# Autodesk Inventor assembly: WheelFront
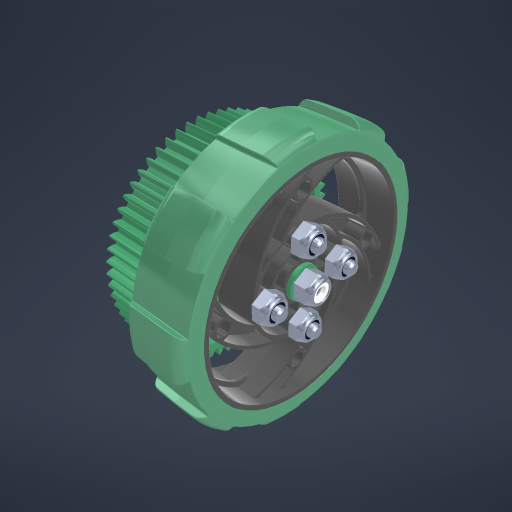
[picture p0: Inventor's stored thumbnail of the model, 512x512]
Saved by Autodesk Inventor 2023 (Build 270158000, 158)
## iProperties
Created: 2022-08-31
Part Number: WheelFront
Document SubType Name: Assembly
Designer: alex
Author: alex
## Documents named in this file (12)
- C:\Users\alex\Documents\GitHub\4067X_spin_up_cad\Chassis\TractionCentre.iam
- C:\Users\alex\Documents\GitHub\4067X_spin_up_cad\Library\Motion\Spacers\Spacer Nylon .375 OD.ipt
- C:\Users\alex\Documents\GitHub\4067X_spin_up_cad\Library\Structure\Hardware\Nut Keps.ipt
- C:\Users\alex\Documents\GitHub\4067X_spin_up_cad\Library\Structure\Hardware\Nut Nylock.ipt
- C:\Users\alex\Documents\GitHub\4067X_spin_up_cad\Library\Structure\Hardware\Screw Steel - Star.ipt
- C:\Users\alex\Documents\GitHub\4067X_spin_up_cad\Library\Structure\Hardware\Screw Steel - Star\SScrew Star Smooth 1.500.ipt
- C:\Users\alex\Documents\GitHub\4067X_spin_up_cad\Library\Structure\Hardware\Nut Thin Nylock.ipt
- C:\Users\alex\Documents\GitHub\4067X_spin_up_cad\Library\Structure\Standoff\Standoff .50.ipt
- C:\Users\alex\Documents\GitHub\4067X_spin_up_cad\Library\Structure\Standoff.ipt
- C:\Users\alex\Documents\GitHub\4067X_spin_up_cad\Library\Motion\Gears\HS 60T Gear, Circle.ipt
- C:\Users\alex\Documents\GitHub\4067X_spin_up_cad\Library\Motion\Wheels\Tractions\3.25 Traction, Circle.ipt
- C:\Users\alex\Documents\GitHub\4067X_spin_up_cad\Library\Motion\Spacers\Spacer Nylon .375 OD\NSpacer .375 OD x .125.ipt
## Components (20 placed, 8 different names)
1. HS 60T Gear, Circle:1 — Insert:7, Insert:8, Insert:15, Insert:16, Insert:17, Insert:19, Insert:21, Insert:23, Insert:25
2. Standoff .50:1 — Insert:7
3. Standoff .50:2 — Insert:8
4. 3.25 Traction, Circle:1 — Insert:14, Insert:26, Insert:27, Insert:28, Insert:29
5. Nut Nylock:1 — Insert:14
6. Nut Keps:1 — Insert:15
7. Standoff .50:3 — Insert:16
8. Standoff .50:4 — Insert:17
9. SScrew Star Smooth 1.500:1
10. NSpacer .375 OD x .125:1 — Insert:19
11. SScrew Star Smooth 1.500:2
12. NSpacer .375 OD x .125:2 — Insert:21
13. SScrew Star Smooth 1.500:3
14. NSpacer .375 OD x .125:3 — Insert:23
15. SScrew Star Smooth 1.500:4
16. NSpacer .375 OD x .125:4 — Insert:25
17. Nut Thin Nylock:3 — Insert:26
18. Nut Thin Nylock:4 — Insert:27
19. Nut Thin Nylock:5 — Insert:28
20. Nut Thin Nylock:6 — Insert:29
## Relationships (18: Insert 18)
- Insert:7: HS 60T Gear, Circle:1 ↔ Standoff .50:1
- Insert:8: HS 60T Gear, Circle:1 ↔ Standoff .50:2
- Insert:14: 3.25 Traction, Circle:1 ↔ Nut Nylock:1
- Insert:15: HS 60T Gear, Circle:1 ↔ Nut Keps:1
- Insert:16: HS 60T Gear, Circle:1 ↔ Standoff .50:3
- Insert:17: HS 60T Gear, Circle:1 ↔ Standoff .50:4
- [Insert]: SScrew Star Smooth 1.500:1 ↔ NSpacer .375 OD x .125:1
- Insert:19: HS 60T Gear, Circle:1 ↔ NSpacer .375 OD x .125:1
- [Insert]: SScrew Star Smooth 1.500:2 ↔ NSpacer .375 OD x .125:2
- Insert:21: HS 60T Gear, Circle:1 ↔ NSpacer .375 OD x .125:2
- [Insert]: SScrew Star Smooth 1.500:3 ↔ NSpacer .375 OD x .125:3
- Insert:23: HS 60T Gear, Circle:1 ↔ NSpacer .375 OD x .125:3
- [Insert]: SScrew Star Smooth 1.500:4 ↔ NSpacer .375 OD x .125:4
- Insert:25: HS 60T Gear, Circle:1 ↔ NSpacer .375 OD x .125:4
- Insert:26: 3.25 Traction, Circle:1 ↔ Nut Thin Nylock:3
- Insert:27: 3.25 Traction, Circle:1 ↔ Nut Thin Nylock:4
- Insert:28: 3.25 Traction, Circle:1 ↔ Nut Thin Nylock:5
- Insert:29: 3.25 Traction, Circle:1 ↔ Nut Thin Nylock:6
## Named parameters: d60_d58_d57 = 0 mm, d72_d60_d58_d57 = 0 mm, d74_d60_d58_d57 = 0 mm, d76_d60_d58_d57 = 0 mm
